# Autodesk Inventor assembly: PIPE ASSEMBLY
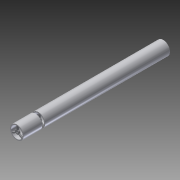
[picture p0: Inventor's stored thumbnail of the model, 180x180]
Saved by Autodesk Inventor 2013 (Build 170138000, 138)
## iProperties
Created: 2013-12-04
Part Number: PIPE ASSEMBLY
Document SubType Name: Assembly
Designer: employee
Author: employee
## Documents named in this file (4)
- C:\Users\employee\Desktop\ConceptFORGE\ConceptFORGE\LISA Simpson\INVENTOR FILES\PIPE ASSEMBLY.iam
- C:\Users\employee\Desktop\ConceptFORGE\ConceptFORGE\LISA Simpson\INVENTOR FILES\_SHORT PIPE.ipt
- C:\Users\employee\Desktop\ConceptFORGE\ConceptFORGE\LISA Simpson\INVENTOR FILES\_LONG PIPE.ipt
- C:\Users\employee\Desktop\ConceptFORGE\ConceptFORGE\LISA Simpson\INVENTOR FILES\ALLIGNER.ipt
## Components (6 placed, 3 different names)
1. _SHORT PIPE:1 — Insert:2, Insert:6
2. _LONG PIPE:1 — Insert:3, Insert:4
3. ALLIGNER:1 — Insert:6
4. ALLIGNER:2 — Insert:2, Insert:5
5. ALLIGNER:3 — Insert:3, Insert:5
6. ALLIGNER:4 — Insert:4
## Relationships (5: Insert 5)
- Insert:2: _SHORT PIPE:1 ↔ ALLIGNER:2
- Insert:3: _LONG PIPE:1 ↔ ALLIGNER:3
- Insert:4: _LONG PIPE:1 ↔ ALLIGNER:4
- Insert:5 (12.5 mm): ALLIGNER:2 ↔ ALLIGNER:3
- Insert:6: _SHORT PIPE:1 ↔ ALLIGNER:1
